# Autodesk Inventor assembly: Helix DLP Z Stage
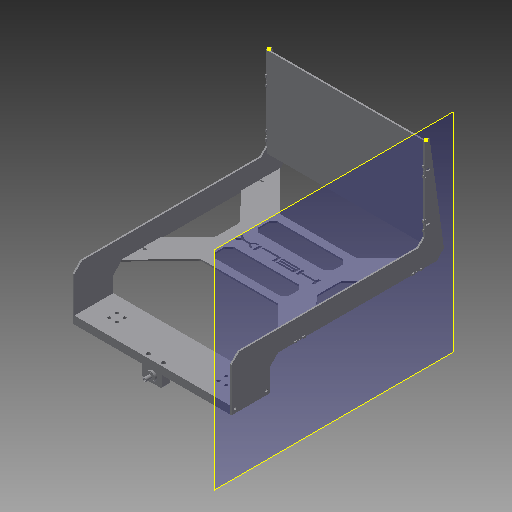
[picture p0: Inventor's stored thumbnail of the model, 512x512]
Saved by Autodesk Inventor 2019 (Build 230136000, 136)
## iProperties
Created: 2020-03-07
Part Number: Helix DLP Z Stage
Document SubType Name: Assembly
Designer: Vijay
Author: Vijay
## Documents named in this file (8)
- C:\Users\Vijay\Documents\CAD Files\Helix DLP\Helix DLP Z Stage.iam
- C:\Users\Vijay\Documents\CAD Files\Helix DLP\Print Platform.ipt
- C:\Users\Vijay\Documents\CAD Files\Helix DLP\Z stage_side.ipt
- C:\Users\Vijay\Documents\CAD Files\Helix DLP\Z stage_brace.ipt
- C:\Users\Vijay\Documents\CAD Files\Helix DLP\Z Stage_Linear Block Holder.ipt
- C:\Users\Vijay\Documents\CAD Files\Helix DLP\mgn12-linear-guide-subassembly-with-configurable-rail-length-1.snapshot.8\MGN12H, LINEAR GUIDE BLOCK.ipt
- C:\Users\Vijay\Documents\CAD Files\Helix DLP\Z Leadcrew Nut Holder.ipt
- C:\Users\Vijay\Documents\CAD Files\Julia Extended Rev19\Julia Chassi(Chamfered)\Julia Chassi(Chamfered)\Julia 3D model\Z Motor Screw.ipt
## Components (9 placed, 7 different names)
1. Print Platform:1 — Flush:1, Mate:1
2. Z stage_side:1 — Flush:1, Flush:2, Flush:3, Flush:4, Flush:10, Flush:13
3. Z stage_side:2 — Flush:2, Flush:3, Mate:1, Flush:5, Flush:6, Flush:11
4. Z stage_brace:1 — Flush:4
5. Z Stage_Linear Block Holder:1 — Flush:5, Flush:6, Flush:9, Mate:2, Flush:12, Flush:14
6. MGN12H, LINEAR GUIDE BLOCK:1 — Flush:7, Flush:8, Flush:11, Mate:2
7. MGN12H, LINEAR GUIDE BLOCK:2 — Flush:7, Flush:8, Flush:9, Flush:10
8. Z Leadcrew Nut Holder:1 — Flush:12, Flush:13, Flush:14, Mate:3, Mate:4, Mate:5
9. Z Motor Screw:1 — Mate:3, Mate:4, Mate:5
## Relationships (19: Flush 14, Mate 5)
- Flush:1: Print Platform:1 ↔ Z stage_side:1
- Flush:2: Z stage_side:1 ↔ Z stage_side:2
- Flush:3: Z stage_side:1 ↔ Z stage_side:2
- Mate:1: Print Platform:1 ↔ Z stage_side:2
- Flush:4: Z stage_side:1 ↔ Z stage_brace:1
- Flush:5: Z stage_side:2 ↔ Z Stage_Linear Block Holder:1
- Flush:6: Z stage_side:2 ↔ Z Stage_Linear Block Holder:1
- Flush:7: MGN12H, LINEAR GUIDE BLOCK:1 ↔ MGN12H, LINEAR GUIDE BLOCK:2
- Flush:8: MGN12H, LINEAR GUIDE BLOCK:1 ↔ MGN12H, LINEAR GUIDE BLOCK:2
- Flush:9 (27.3 mm): Z Stage_Linear Block Holder:1 ↔ MGN12H, LINEAR GUIDE BLOCK:2
- Flush:10 (50 mm): Z stage_side:1 ↔ MGN12H, LINEAR GUIDE BLOCK:2
- Flush:11 (50 mm): Z stage_side:2 ↔ MGN12H, LINEAR GUIDE BLOCK:1
- Mate:2: Z Stage_Linear Block Holder:1 ↔ MGN12H, LINEAR GUIDE BLOCK:1
- Flush:12: Z Stage_Linear Block Holder:1 ↔ Z Leadcrew Nut Holder:1
- Flush:13 (179 mm): Z stage_side:1 ↔ Z Leadcrew Nut Holder:1
- Flush:14: Z Stage_Linear Block Holder:1 ↔ Z Leadcrew Nut Holder:1
- Mate:3: Z Leadcrew Nut Holder:1 ↔ Z Motor Screw:1
- Mate:4: Z Leadcrew Nut Holder:1 ↔ Z Motor Screw:1
- Mate:5: Z Leadcrew Nut Holder:1 ↔ Z Motor Screw:1
